# Autodesk Inventor assembly: CDAS16X10
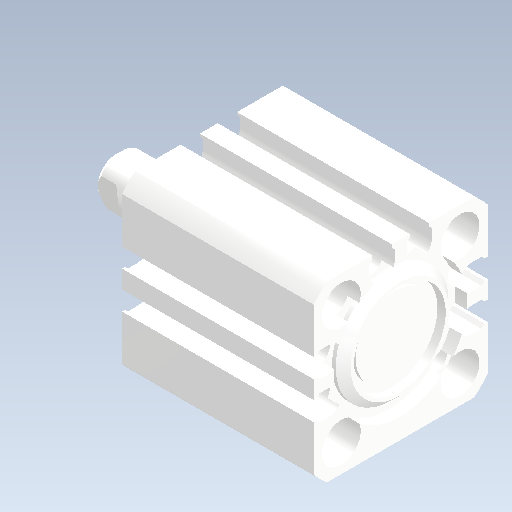
[picture p0: Inventor's stored thumbnail of the model, 512x512]
Saved by Autodesk Inventor 2021.2 (Build 252289000, 289)
## iProperties
Created: 2016-07-24
Part Number: CDAS16X10
Document SubType Name: Assembly
Designer: yuta2
Mass: 65.4494 g
Surface Area: 122.216 cm^2
Volume: 18.1432 cm^3
Density: 3.60738 g/cm^3
Sending System: spGate
Preprocessor: spGate 11.3.7
Title: HCDAS16X10.stp
## Documents named in this file (3)
- C:\Users\Hagihara Yuya\Documents\GrabCAD\NHK2021\BasicParts\よく使う部品（萩原）\AirCylinder\CDAS16X10\CDAS16X10.iam
- C:\Users\Hagihara Yuya\Documents\GrabCAD\NHK2021\BasicParts\よく使う部品（萩原）\AirCylinder\CDAS16X10\HCDAS16X10-prt0.ipt
- C:\Users\Hagihara Yuya\Documents\GrabCAD\NHK2021\BasicParts\よく使う部品（萩原）\AirCylinder\CDAS16X10\HCDAS16X10-prt1.ipt
## Components (2 placed, 2 different names)
1. HCDAS16X10-prt0 — 円柱状:1
2. HCDAS16X10-prt1 — 円柱状:1
## Relationships (1: CylindricalJoint 1)
- 円柱状:1 [CylindricalJoint]: HCDAS16X10-prt0 ↔ HCDAS16X10-prt1
